# Autodesk Inventor assembly: Finger
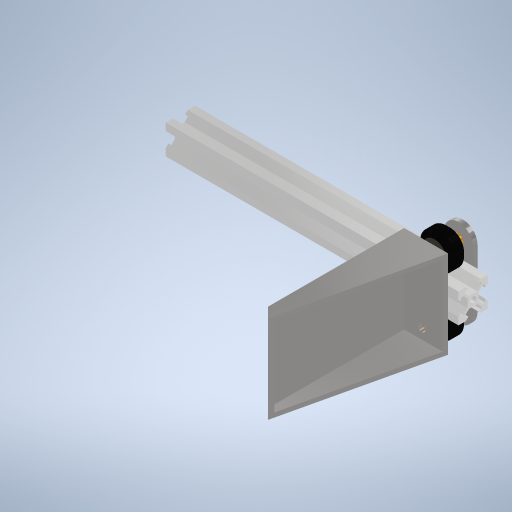
[picture p0: Inventor's stored thumbnail of the model, 512x512]
Saved by Autodesk Inventor 2024.2 (Build 282272000, 272)
## iProperties
Created: 2025-04-11
Part Number: Finger
Document SubType Name: Assembly
Designer: Admin
Author: Admin
## Documents named in this file (5)
- C:\Users\Admin\Documents\GitHub\GripperPropuesto\Assemblies\Finger.iam
- C:\Users\Admin\Documents\GitHub\GripperPropuesto\Assemblies\BearingWithInsert.iam
- C:\Users\Admin\Documents\GitHub\GripperPropuesto\AuxiliarPieces\FingerSupport\FingerSupport.ipt
- C:\Users\Admin\Documents\GitHub\GripperPropuesto\AuxiliarPieces\AluminumProfile\AP20x20.ipt
- C:\Users\Admin\Documents\GitHub\GripperPropuesto\AuxiliarPieces\Claw\Claw.ipt
## Components (5 placed, 4 different names)
1. BearingWithInsert:1 [sub-assembly] — Tangent:1, Tangent:2, Mate:1, Mate:2, Mate:6
2. BearingWithInsert:2 [sub-assembly] — Tangent:3, Tangent:4, Mate:3, Mate:4, Mate:5, Mate:7
3. AP20x20:1 — Tangent:1, Tangent:2, Tangent:3, Tangent:4
4. FingerSupport:1 — Mate:1, Mate:2, Mate:3, Mate:4
5. Claw:1 — Mate:5, Mate:6, Mate:7
## Relationships (11: Mate 7, Tangent 4)
- Tangent:1: BearingWithInsert:1 ↔ AP20x20:1
- Tangent:2: BearingWithInsert:1 ↔ AP20x20:1
- Tangent:3: BearingWithInsert:2 ↔ AP20x20:1
- Tangent:4: BearingWithInsert:2 ↔ AP20x20:1
- Mate:1: BearingWithInsert:1 ↔ FingerSupport:1
- Mate:2: BearingWithInsert:1 ↔ FingerSupport:1
- Mate:3: BearingWithInsert:2 ↔ FingerSupport:1
- Mate:4: BearingWithInsert:2 ↔ FingerSupport:1
- Mate:5: BearingWithInsert:2 ↔ Claw:1
- Mate:6: BearingWithInsert:1 ↔ Claw:1
- Mate:7: BearingWithInsert:2 ↔ Claw:1
